# Autodesk Inventor assembly: Trunk_neck_frame_AND_Trunk_shoulder_frame_WearingImage
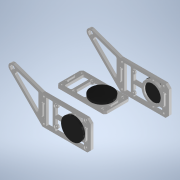
[picture p0: Inventor's stored thumbnail of the model, 180x180]
Saved by Autodesk Inventor 2020.4 (Build 244396000, 396)
## iProperties
Created: 2022-03-16
Part Number: Trunk_neck_frame_AND_Trunk_shoulder_frame_WearingImage
Document SubType Name: Assembly
Designer: Masato Kubotera
Author: Masato Kubotera
## Documents named in this file (5)
- C:\Users\Masato\Documents\Inventor\CIT Brains_Inventor\SUSTAINA-OP\SandBlastingJig\Trunk_neck_frame_AND_Trunk_shoulder_frame_WearingImage.iam
- C:\Users\Masato\Documents\Inventor\CIT Brains_Inventor\SUSTAINA-OP\UpperBody\Trunk\Trunk_neck_frame.ipt
- C:\Users\Masato\Documents\Inventor\CIT Brains_Inventor\SUSTAINA-OP\UpperBody\Trunk\Trunk_shoulder_frame_MIR.ipt
- C:\Users\Masato\Documents\Inventor\CIT Brains_Inventor\SUSTAINA-OP\SandBlastingJig\Trunk_neck_frame_AND_Trunk_shoulder_frame_SandBlastingJig.ipt
- C:\Users\Masato\Documents\Inventor\CIT Brains_Inventor\SUSTAINA-OP\UpperBody\Trunk\Trunk_shoulder_frame.ipt
## Components (6 placed, 4 different names)
1. Trunk_neck_frame:1 — 挿入:2
2. Trunk_shoulder_frame:1 — 挿入:3
3. Trunk_shoulder_frame_MIR:1 — 挿入:4
4. Trunk_neck_frame_AND_Trunk_shoulder_frame_SandBlastingJig:1 — 挿入:2
5. Trunk_neck_frame_AND_Trunk_shoulder_frame_SandBlastingJig:2 — 挿入:4
6. Trunk_neck_frame_AND_Trunk_shoulder_frame_SandBlastingJig:3 — 挿入:3
## Relationships (3: Insert 3)
- 挿入:2 [Insert]: Trunk_neck_frame:1 ↔ Trunk_neck_frame_AND_Trunk_shoulder_frame_SandBlastingJig:1
- 挿入:3 [Insert]: Trunk_shoulder_frame:1 ↔ Trunk_neck_frame_AND_Trunk_shoulder_frame_SandBlastingJig:3
- 挿入:4 [Insert]: Trunk_shoulder_frame_MIR:1 ↔ Trunk_neck_frame_AND_Trunk_shoulder_frame_SandBlastingJig:2
